# Autodesk Inventor assembly: Ensamble caja aleja
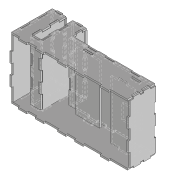
[picture p0: Inventor's stored thumbnail of the model, 180x180]
Saved by Autodesk Inventor 2022 (Build 260153000, 153)
## iProperties
Created: 2022-06-21
Part Number: Ensamble caja aleja
Document SubType Name: Assembly
Designer: ADMIN
Author: ADMIN
## Documents named in this file (10)
- C:\Users\ADMIN\Documents\piezas varias\Caja Alejandra\Ensamble caja aleja.iam
- C:\Users\ADMIN\Documents\piezas varias\Caja Alejandra\Frontal.ipt
- C:\Users\ADMIN\Documents\piezas varias\Caja Alejandra\Superior 1.ipt
- C:\Users\ADMIN\Documents\piezas varias\Caja Alejandra\Sup´2.ipt
- C:\Users\ADMIN\Documents\piezas varias\Caja Alejandra\Lat 1.ipt
- C:\Users\ADMIN\Documents\piezas varias\Caja Alejandra\Lat 2.ipt
- C:\Users\ADMIN\Documents\piezas varias\Caja Alejandra\Lat 3.ipt
- C:\Users\ADMIN\Documents\piezas varias\Caja Alejandra\Superior 2.ipt
- C:\Users\ADMIN\Documents\piezas varias\Caja Alejandra\LAT 4.ipt
- C:\Users\ADMIN\Documents\piezas varias\Caja Alejandra\piso medio.ipt
## Components (13 placed, 9 different names)
1. Frontal:1 — Flush:1, Flush:2
2. Frontal:2 — Flush:1, Flush:2, Flush:3, Flush:4, Flush:5, Mate:1, Flush:6, Flush:7, Flush:8, Flush:9, Flush:10, Flush:11, Flush:12, Flush:13, Flush:14, Mate:2, Flush:15, Flush:16, Flush:17, Flush:18, Flush:19
3. Superior 1:1 — Flush:3, Flush:4
4. Sup´2:1 — Flush:5, Mate:1
5. Lat 1:1 — Flush:6, Flush:7
6. Superior 1:2 — Flush:8, Flush:9
7. Lat 2:1 — Flush:10, Flush:11
8. Lat 3:1 — Flush:12, Flush:13
9. Superior 2:1 — Flush:14, Mate:2
10. LAT 4:1 — Flush:15, Flush:16
11. Lat 3:2 — Flush:17, Flush:18
12. piso medio:1 — Flush:19
13. piso medio:2
## Relationships (21: Flush 19, Mate 2)
- Flush:1: Frontal:1 ↔ Frontal:2
- Flush:2: Frontal:1 ↔ Frontal:2
- Flush:3: Frontal:2 ↔ Superior 1:1
- Flush:4: Frontal:2 ↔ Superior 1:1
- Flush:5: Frontal:2 ↔ Sup´2:1
- Mate:1: Frontal:2 ↔ Sup´2:1
- Flush:6: Frontal:2 ↔ Lat 1:1
- Flush:7: Frontal:2 ↔ Lat 1:1
- Flush:8: Frontal:2 ↔ Superior 1:2
- Flush:9: Frontal:2 ↔ Superior 1:2
- Flush:10: Frontal:2 ↔ Lat 2:1
- Flush:11: Frontal:2 ↔ Lat 2:1
- Flush:12: Frontal:2 ↔ Lat 3:1
- Flush:13: Frontal:2 ↔ Lat 3:1
- Flush:14: Frontal:2 ↔ Superior 2:1
- Mate:2: Frontal:2 ↔ Superior 2:1
- Flush:15: Frontal:2 ↔ LAT 4:1
- Flush:16: Frontal:2 ↔ LAT 4:1
- Flush:17: Frontal:2 ↔ Lat 3:2
- Flush:18: Frontal:2 ↔ Lat 3:2
- Flush:19: Frontal:2 ↔ piso medio:1
